# Autodesk Inventor assembly: stackup
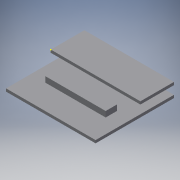
[picture p0: Inventor's stored thumbnail of the model, 180x180]
Saved by Autodesk Inventor 2018 (Build 220112000, 112)
## iProperties
Created: 2017-12-03
Part Number: stackup
Document SubType Name: Assembly
Designer: Cole Tucker
Author: Cole Tucker
## Documents named in this file (3)
- C:\Users\Cole Tucker\OneDrive\FRC-mxpProject\Cad\inventor\stackup.iam
- C:\Users\Cole Tucker\OneDrive\FRC-mxpProject\Cad\inventor\mainboard.ipt
- C:\Users\Cole Tucker\OneDrive\FRC-mxpProject\Cad\inventor\powerreg.ipt
## Components (2 placed, 2 different names)
1. mainboard:1 — Flush:1, Flush:2, Flush:3
2. powerreg:1 — Flush:1, Flush:2, Flush:3
## Relationships (3: Flush 3)
- Flush:1: mainboard:1 ↔ powerreg:1
- Flush:2: mainboard:1 ↔ powerreg:1
- Flush:3 (-12.7 mm): mainboard:1 ↔ powerreg:1
